# Autodesk Inventor assembly: MasterCtrlCase
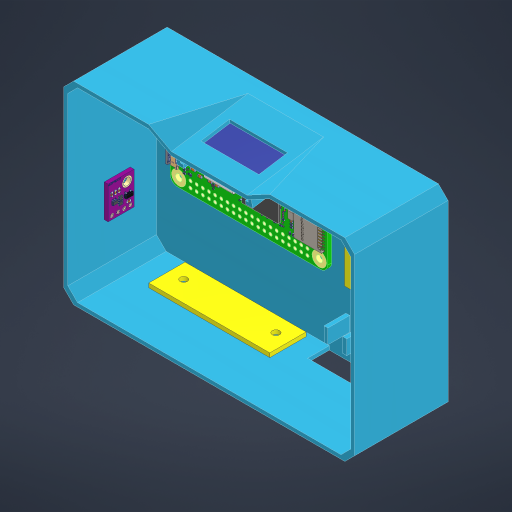
[picture p0: Inventor's stored thumbnail of the model, 512x512]
Saved by Autodesk Inventor 2024.2 (Build 282272000, 272)
## iProperties
Created: 2024-06-03
Part Number: MasterCtrlCase
Document SubType Name: Assembly
Designer: simon
Author: simon
## Documents named in this file (7)
- C:\Users\simon\Documents\Repositories\GrowBox\hardware\MasterCtrlCase\MasterCtrlCase.iam
- C:\Users\simon\Documents\Repositories\GrowBox\hardware\MasterCtrlCase\BasePlate.ipt
- C:\Users\simon\Documents\Repositories\GrowBox\hardware\MasterCtrlCase\step\Raspberry Pi Zero 2 W\Raspberry Pi Zero 2 W.iam
- C:\Users\simon\Documents\Repositories\GrowBox\hardware\MasterCtrlCase\step\Weewooday I2C OLED 0.98” 128x64\Weewooday I2C OLED 0.98” 128x64.iam
- C:\Users\simon\Documents\Repositories\GrowBox\hardware\MasterCtrlCase\293D.ipt
- C:\Users\simon\Documents\Repositories\GrowBox\hardware\MasterCtrlCase\step\GY-BME280\GY-BME280.ipt
- C:\Users\simon\Documents\Repositories\GrowBox\hardware\MasterCtrlCase\DeviceConnector.ipt
## Components (6 placed, 6 different names)
1. BasePlate:1 — Mate:1, Mate:2, Flush:1, Flush:2, Flush:3, Flush:4, Flush:6, Mate:3, Flush:8, Mate:5
2. Raspberry Pi Zero 2 W:1 [sub-assembly] — Flush:2, Flush:8
3. Weewooday I2C OLED 0.98” 128x64:1 [sub-assembly] — Flush:5, Flush:7
4. 293D:1 — Flush:3, Mate:3
5. GY-BME280:1 — Mate:4, Flush:9
6. DeviceConnector:1 — Mate:5, Flush:10, Flush:11
## Relationships (16: Flush 11, Mate 5)
- Mate:1: BasePlate:1
- Mate:2: BasePlate:1
- Flush:1: BasePlate:1
- Flush:2 (4 mm): BasePlate:1 ↔ Raspberry Pi Zero 2 W:1
- Flush:3 (4 mm): BasePlate:1 ↔ 293D:1
- Flush:4: BasePlate:1
- Flush:5 (15.8 mm): Weewooday I2C OLED 0.98” 128x64:1
- Flush:6: BasePlate:1
- Flush:7 (26.4 mm): Weewooday I2C OLED 0.98” 128x64:1
- Mate:3 (37.1 mm): BasePlate:1 ↔ 293D:1
- Flush:8 (77.4 mm): BasePlate:1 ↔ Raspberry Pi Zero 2 W:1
- Mate:4 (-115 mm): GY-BME280:1
- Flush:9 (20 mm): GY-BME280:1
- Mate:5: BasePlate:1 ↔ DeviceConnector:1
- Flush:10 (-105 mm): DeviceConnector:1
- Flush:11 (3.6 mm): DeviceConnector:1
